# Autodesk Inventor assembly: Assembly
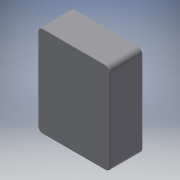
[picture p0: Inventor's stored thumbnail of the model, 180x180]
Saved by Autodesk Inventor 2016 (Build 200138000, 138)
## iProperties
Created: 2016-03-25
Part Number: Assembly
Document SubType Name: Assembly
Designer: Paschalis
Author: Paschalis
## Documents named in this file (3)
- C:\Users\Paschalis\Documents\eagle\Measuring-PCB\3D\Assembly.iam
- C:\Users\Paschalis\Documents\eagle\Measuring-PCB\3D\box_base.ipt
- C:\Users\Paschalis\Documents\eagle\Measuring-PCB\3D\board2.brd.iam
## Components (2 placed, 2 different names)
1. box_base:1 — Mate:1, Mate:2, Mate:3
2. board2.brd:1 [sub-assembly] — Mate:1, Mate:2, Mate:3
## Relationships (3: Mate 3)
- Mate:1 (5 mm): box_base:1 ↔ board2.brd:1
- Mate:2 (20 mm): box_base:1 ↔ board2.brd:1
- Mate:3 (10 mm): box_base:1 ↔ board2.brd:1
